# Autodesk Inventor assembly: ArcadeController
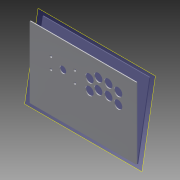
[picture p0: Inventor's stored thumbnail of the model, 180x180]
Saved by Autodesk Inventor 2013 (Build 170138000, 138)
## iProperties
Created: 2013-02-02
Part Number: ArcadeController
Document SubType Name: Assembly
Designer: xylzlyx
Author: xylzlyx
## Documents named in this file (3)
- C:\dev\pewpew\assemblies\ArcadeController.iam
- C:\dev\pewpew\parts\Panel_top.ipt
- C:\dev\pewpew\parts\Panel_bottom.ipt
## Components (2 placed, 2 different names)
1. TopPanel:1 — Flush:1, Mate:1
2. BottomPanel:1 — Flush:1, Mate:1
## Relationships (2: Flush 1, Mate 1)
- Flush:1: TopPanel:1 ↔ BottomPanel:1
- Mate:1: TopPanel:1 ↔ BottomPanel:1
